# Autodesk Inventor assembly: j2
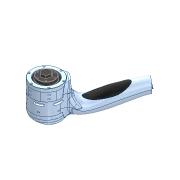
[picture p0: Inventor's stored thumbnail of the model, 180x180]
Saved by Autodesk Inventor 2021 (Build 250183000, 183)
## iProperties
Created: 2020-08-05
Part Number: j2
Document SubType Name: Assembly
Designer: Derm
Mass: 963.665 g
Surface Area: 3780.03 cm^2
Volume: 901.378 cm^3
Density: 1.0691 g/cm^3
Author: Derm
## Documents named in this file (19)
- C:\Users\Derm\roboticArm\hardware\v9\j2.iam
- C:\Users\Derm\roboticArm\hardware\v9\100kv motor.ipt
- C:\Users\Derm\roboticArm\hardware\v9\j0RingGear.ipt
- C:\Users\Derm\roboticArm\hardware\v9\6823-2RS.ipt
- C:\Users\Derm\roboticArm\hardware\v9\Healical Gear (12R@0.00).ipt
- C:\Users\Derm\roboticArm\hardware\v9\Planet Carrier Front BEEFY EXTENDO.ipt
- C:\Users\Derm\roboticArm\hardware\v9\Planet Carrier Back.ipt
- C:\Users\Derm\roboticArm\hardware\v9\Healical Gear (24L@15.00).ipt
- C:\Users\Derm\roboticArm\hardware\v9\6153K15.ipt
- C:\Users\Derm\roboticArm\hardware\v9\93600A608.ipt
- C:\Users\Derm\roboticArm\hardware\v9\100kvMotorEncoderShaft.ipt
- C:\Users\Derm\roboticArm\hardware\v9\AMT-102-Wide-Base-REV-J.ipt
- C:\Users\Derm\roboticArm\hardware\v9\AMT-102-Top-Cover-REV-H.ipt
- C:\Users\Derm\roboticArm\hardware\v9\Front Plate.ipt
- C:\Users\Derm\roboticArm\hardware\v9\AMT102Mount.ipt
- C:\Users\Derm\roboticArm\hardware\v9\j2HousingV2.ipt
- C:\Users\Derm\roboticArm\hardware\v9\2020 Aluminium Extrusion T-Slot lower arm.ipt
- C:\Users\Derm\roboticArm\hardware\v9\j2Base.ipt
- C:\Users\Derm\roboticArm\hardware\v9\lowerArmMidV2.ipt
## Components (28 placed, 18 different names)
1. 100kv motor:1 — Mate:3, Mate:4, Mate:5, Mate:12, Mate:37, Mate:38, Mate:49, Mate:50
2. j0RingGear:1 — Mate:42, Mate:43, Mate:44, Flush:12, Mate:46, Mate:47, Mate:48, Mate:63
3. 6823-2RS:1 — Mate:12, Mate:13, Mate:14, Mate:15, Mate:16
4. Healical Gear (12R@0.00):3 — Mate:3, Mate:4, Mate:5
5. 6823-2RS:2 — Mate:14, Mate:36, Mate:46
6. Planet Carrier Front BEEFY EXTENDO:1 — Mate:15, Mate:16, Mate:17, Mate:18, Mate:19, Mate:45
7. Planet Carrier Back:1 — Mate:17, Mate:18, Mate:19, Mate:20, Mate:30, Mate:31, Mate:32, Mate:33, Mate:34, Mate:35, Mate:36
8. Healical Gear (24L@15.00):1 — Mate:20, Mate:21, Mate:22, Flush:2, Flush:3, Flush:4, Mate:35
9. 6153K15:1 — Mate:21, Flush:3, Mate:23
10. 6153K15:2 — Mate:22, Flush:2
11. 93600A608:1 — Mate:23, Flush:4, Mate:30
12. Healical Gear (24L@15.00):2 — Mate:33
13. 6153K15:3
14. 6153K15:4
15. 93600A608:2 — Mate:31
16. Healical Gear (24L@15.00):3 — Mate:34
17. 6153K15:5
18. 6153K15:6
19. 93600A608:3 — Mate:32
20. 100kvMotorEncoderShaft:1 — Mate:37, Mate:38, Mate:41, Mate:64
21. AMT-102-Wide-Base-REV-J:1 — Mate:39, Mate:40, Mate:41, Flush:11, Mate:66, Mate:52
22. AMT-102-Top-Cover-REV-H:1 — Mate:39, Mate:40, Flush:11
23. Front Plate:1 — Mate:42, Mate:43, Mate:44, Mate:45
24. j2HousingV2:1 — Mate:47, Mate:48, Mate:49, Mate:50, Flush:13, Mate:66, Mate:55, Mate:58, Mate:61, Mate:62, Mate:63, Mate:65, Flush:15, Mate:67, Mate:68, Flush:17, Flush:18
25. AMT102Mount:1 — Flush:13, Mate:52, Mate:64, Mate:65
26. j2Base:1 — Mate:55, Mate:58, Mate:61, Mate:62, Mate:67, Flush:16
27. 2020 Aluminium Extrusion T-Slot lower arm:1 — Flush:15, Flush:16, Flush:19, Flush:20
28. lowerArmMidV2:1 — Mate:68, Flush:17, Flush:18, Flush:19, Flush:20
## Relationships (71: Mate 53, Flush 18)
- Mate:3: 100kv motor:1 ↔ Healical Gear (12R@0.00):3
- Mate:4: 100kv motor:1 ↔ Healical Gear (12R@0.00):3
- Mate:5: 100kv motor:1 ↔ Healical Gear (12R@0.00):3
- Mate:12: 100kv motor:1 ↔ 6823-2RS:1
- Mate:13: 6823-2RS:1
- Mate:14: 6823-2RS:1 ↔ 6823-2RS:2
- Mate:15: 6823-2RS:1 ↔ Planet Carrier Front BEEFY EXTENDO:1
- Mate:16: 6823-2RS:1 ↔ Planet Carrier Front BEEFY EXTENDO:1
- Mate:17: Planet Carrier Front BEEFY EXTENDO:1 ↔ Planet Carrier Back:1
- Mate:18: Planet Carrier Front BEEFY EXTENDO:1 ↔ Planet Carrier Back:1
- Mate:19: Planet Carrier Front BEEFY EXTENDO:1 ↔ Planet Carrier Back:1
- Mate:20: Planet Carrier Back:1 ↔ Healical Gear (24L@15.00):1
- Mate:21: Healical Gear (24L@15.00):1 ↔ 6153K15:1
- Mate:22: Healical Gear (24L@15.00):1 ↔ 6153K15:2
- Flush:2: Healical Gear (24L@15.00):1 ↔ 6153K15:2
- Flush:3: Healical Gear (24L@15.00):1 ↔ 6153K15:1
- Mate:23: 6153K15:1 ↔ 93600A608:1
- Flush:4 (-10.795 mm): Healical Gear (24L@15.00):1 ↔ 93600A608:1
- [Mate]: Healical Gear (24L@15.00):2 ↔ 6153K15:3
- [Mate]: Healical Gear (24L@15.00):2 ↔ 6153K15:4
- [Flush]: Healical Gear (24L@15.00):2 ↔ 6153K15:4
- [Flush]: Healical Gear (24L@15.00):2 ↔ 6153K15:3
- [Mate]: 6153K15:3 ↔ 93600A608:2
- [Flush] (-10.795 mm): Healical Gear (24L@15.00):2 ↔ 93600A608:2
- [Mate]: Healical Gear (24L@15.00):3 ↔ 6153K15:5
- [Mate]: Healical Gear (24L@15.00):3 ↔ 6153K15:6
- [Flush]: Healical Gear (24L@15.00):3 ↔ 6153K15:6
- [Flush]: Healical Gear (24L@15.00):3 ↔ 6153K15:5
- [Mate]: 6153K15:5 ↔ 93600A608:3
- [Flush] (-10.795 mm): Healical Gear (24L@15.00):3 ↔ 93600A608:3
- Mate:30: Planet Carrier Back:1 ↔ 93600A608:1
- Mate:31: Planet Carrier Back:1 ↔ 93600A608:2
- Mate:32: Planet Carrier Back:1 ↔ 93600A608:3
- Mate:33: Planet Carrier Back:1 ↔ Healical Gear (24L@15.00):2
- Mate:34: Planet Carrier Back:1 ↔ Healical Gear (24L@15.00):3
- Mate:35: Planet Carrier Back:1 ↔ Healical Gear (24L@15.00):1
- Mate:36: 6823-2RS:2 ↔ Planet Carrier Back:1
- Mate:37: 100kv motor:1 ↔ 100kvMotorEncoderShaft:1
- Mate:38 (0.5 mm): 100kv motor:1 ↔ 100kvMotorEncoderShaft:1
- Mate:39: AMT-102-Wide-Base-REV-J:1 ↔ AMT-102-Top-Cover-REV-H:1
- Mate:40: AMT-102-Wide-Base-REV-J:1 ↔ AMT-102-Top-Cover-REV-H:1
- Mate:41: 100kvMotorEncoderShaft:1 ↔ AMT-102-Wide-Base-REV-J:1
- Flush:11: AMT-102-Wide-Base-REV-J:1 ↔ AMT-102-Top-Cover-REV-H:1
- Mate:42: j0RingGear:1 ↔ Front Plate:1
- Mate:43: j0RingGear:1 ↔ Front Plate:1
- Mate:44: j0RingGear:1 ↔ Front Plate:1
- Flush:12: j0RingGear:1
- Mate:45: Planet Carrier Front BEEFY EXTENDO:1 ↔ Front Plate:1
- Mate:46: j0RingGear:1 ↔ 6823-2RS:2
- Mate:47: j0RingGear:1 ↔ j2HousingV2:1
- Mate:48: j0RingGear:1 ↔ j2HousingV2:1
- Mate:49: 100kv motor:1 ↔ j2HousingV2:1
- Mate:50: 100kv motor:1 ↔ j2HousingV2:1
- Flush:13: j2HousingV2:1 ↔ AMT102Mount:1
- Mate:66: AMT-102-Wide-Base-REV-J:1 ↔ j2HousingV2:1
- Mate:52: AMT-102-Wide-Base-REV-J:1 ↔ AMT102Mount:1
- Mate:55: j2HousingV2:1 ↔ j2Base:1
- Mate:58: j2HousingV2:1 ↔ j2Base:1
- Mate:61: j2HousingV2:1 ↔ j2Base:1
- Mate:62: j2HousingV2:1 ↔ j2Base:1
- Mate:63: j0RingGear:1 ↔ j2HousingV2:1
- Mate:64: 100kvMotorEncoderShaft:1 ↔ AMT102Mount:1
- Mate:65: j2HousingV2:1 ↔ AMT102Mount:1
- Flush:15 (-10 mm): j2HousingV2:1 ↔ 2020 Aluminium Extrusion T-Slot lower arm:1
- Mate:67: j2HousingV2:1 ↔ j2Base:1
- Flush:16: j2Base:1 ↔ 2020 Aluminium Extrusion T-Slot lower arm:1
- Mate:68: j2HousingV2:1 ↔ lowerArmMidV2:1
- Flush:17: j2HousingV2:1 ↔ lowerArmMidV2:1
- Flush:18: j2HousingV2:1 ↔ lowerArmMidV2:1
- Flush:19: 2020 Aluminium Extrusion T-Slot lower arm:1 ↔ lowerArmMidV2:1
- Flush:20: 2020 Aluminium Extrusion T-Slot lower arm:1 ↔ lowerArmMidV2:1
## Named parameters: d29_d24 = 0 mm, d30_d25 = 0 mm, d31_d26 = 0 mm, d32_d27 = 0 mm, d33_d28 = -10.795 mm, d34_d23 = 0 mm, d35_d24 = 0 mm, d36_d25 = 0 mm, d37_d26 = 0 mm, d38_d27 = 0 mm, d39_d28 = -10.795 mm, d40_d23 = 0 mm
